# Autodesk Inventor assembly: bearings_MIR
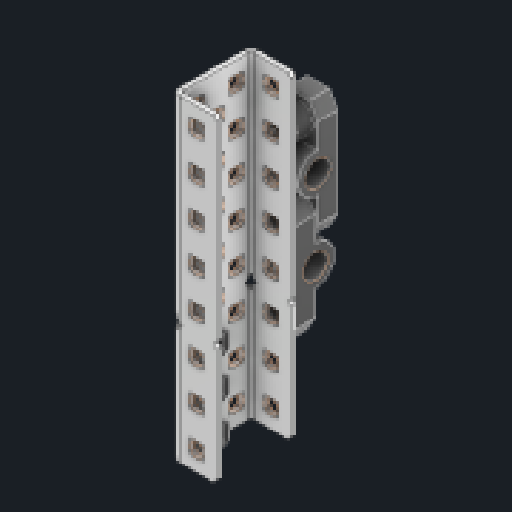
[picture p0: Inventor's stored thumbnail of the model, 512x512]
Saved by Autodesk Inventor 2024 (Build 280153000, 153)
## iProperties
Created: 2023-08-16
Part Number: bearings_MIR
Document SubType Name: Assembly
Designer: avere
Author: avere
## Documents named in this file (11)
- D:\vex_robotics\hardware\cad\scrap_v0.1\catapult\mirrored_parts\bearings_MIR.iam
- D:\vex_robotics\hardware\cad\scrap_v0.1\catapult\mirrored_parts\Bearing Flat Low Profile_MIR.ipt
- D:\vex_robotics\hardware\cad\scrap_v0.1\catapult\mirrored_parts\HS Pillow Bearing Block_MIR.ipt
- D:\vex_robotics\hardware\cad\VEX-CAD-Inventor-1.41\Structure\Hardware\Nut Nylon\Nut Nylon - White.ipt
- D:\vex_robotics\hardware\cad\VEX-CAD-Inventor-1.41\Structure\Hardware\Nut Nylon.ipt
- D:\vex_robotics\hardware\cad\VEX-CAD-Inventor-1.41\Motion\Spacers\Spacer Nylon .375 OD.ipt
- D:\vex_robotics\hardware\cad\VEX-CAD-Inventor-1.41\Motion\Spacers\Spacer Nylon .375 OD\NSpacer .375 OD x .250.ipt
- D:\vex_robotics\hardware\cad\VEX-CAD-Inventor-1.41\Motion\Spacers\Washer Steel\SWasher .375 OD x .062500.ipt
- D:\vex_robotics\hardware\cad\VEX-CAD-Inventor-1.41\Motion\Spacers\Washer Steel.ipt
- D:\vex_robotics\hardware\cad\VEX-CAD-Inventor-1.41\Motion\Spacers\Washer Steel\SWasher .375 OD x .015625.ipt
- D:\vex_robotics\hardware\cad\VEX-CAD-Inventor-1.41\Structure\C Channel\Aluminum 1x2x1\Alu C 1x2x1x8.ipt
## Components (8 placed, 7 different names)
1. Bearing Flat Low Profile_MIR:1 — Insert:10, Mate:6
2. HS Pillow Bearing Block_MIR:1 — Mate:3, Insert:5, Insert:9, Mate:4
3. HS Pillow Bearing Block_MIR:2 — Insert:4, Mate:3, Insert:5
4. Nut Nylon - White:1 — Insert:4, Insert:6
5. NSpacer .375 OD x .250:2 — Insert:6, Insert:8
6. SWasher .375 OD x .062500:1 — Insert:7, Mate:5
7. SWasher .375 OD x .015625:2 — Insert:7, Insert:8
8. Alu C 1x2x1x8:1 — Insert:9, Mate:4, Mate:5, Insert:10, Mate:6
## Relationships (11: Insert 7, Mate 4)
- Insert:4: HS Pillow Bearing Block_MIR:2 ↔ Nut Nylon - White:1
- Mate:3: HS Pillow Bearing Block_MIR:1 ↔ HS Pillow Bearing Block_MIR:2
- Insert:5 (9.525 mm): HS Pillow Bearing Block_MIR:1 ↔ HS Pillow Bearing Block_MIR:2
- Insert:6: Nut Nylon - White:1 ↔ NSpacer .375 OD x .250:2
- Insert:7: SWasher .375 OD x .062500:1 ↔ SWasher .375 OD x .015625:2
- Insert:8: NSpacer .375 OD x .250:2 ↔ SWasher .375 OD x .015625:2
- Insert:9: HS Pillow Bearing Block_MIR:1 ↔ Alu C 1x2x1x8:1
- Mate:4: HS Pillow Bearing Block_MIR:1 ↔ Alu C 1x2x1x8:1
- Mate:5: SWasher .375 OD x .062500:1 ↔ Alu C 1x2x1x8:1
- Insert:10: Bearing Flat Low Profile_MIR:1 ↔ Alu C 1x2x1x8:1
- Mate:6: Bearing Flat Low Profile_MIR:1 ↔ Alu C 1x2x1x8:1
